# Autodesk Inventor assembly: carriage_assembly
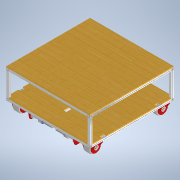
[picture p0: Inventor's stored thumbnail of the model, 180x180]
Saved by Autodesk Inventor 2021.3 (Build 253353000, 353)
## iProperties
Created: 2023-04-09
Part Number: carriage_assembly
Document SubType Name: Assembly
Designer: nxf77172
_SolveAssemblyDoc: Frame Generator Solve Assembly
_Version: 15.0.0
Author: nxf77172
## Documents named in this file (7)
- C:\Users\nxf77172\Desktop\mechanical_cleaned\custom_parts\carriage_assembly.iam
- C:\Users\nxf77172\Desktop\mechanical_cleaned\custom_parts\frame\frame_bottom.iam
- C:\Users\nxf77172\Desktop\mechanical_cleaned\custom_parts\drivetrain\drivetrain_assembly.iam
- C:\Users\nxf77172\Desktop\mechanical_cleaned\custom_parts\Bottom_Plate.ipt
- C:\Users\nxf77172\Desktop\mechanical_cleaned\custom_parts\frame\vertical_struts_frame.ipt
- C:\Users\nxf77172\Desktop\mechanical_cleaned\custom_parts\carriage_assembly\Frame\vertical_frame.iam
- C:\Users\nxf77172\Desktop\mechanical_cleaned\custom_parts\frame\frame_top.iam
## Components (9 placed, 6 different names)
1. frame_bottom:1 [sub-assembly] — Mate:1, Angle:1, Flush:1, Mate:2, Mate:3, Mate:4, Mate:5, Angle:2, Mate:7, Mate:8, Mate:10, Mate:11, Angle:3, Mate:12, Mate:13, Mate:15, Mate:16, Mate:20, Flush:2
2. drivetrain_assembly:1 [sub-assembly] — Mate:2, Mate:3, Mate:6
3. drivetrain_assembly:2 [sub-assembly] — Mate:7, Mate:8, Mate:9
4. drivetrain_assembly:3 [sub-assembly] — Mate:12, Mate:13, Mate:14
5. drivetrain_assembly:4 [sub-assembly] — Mate:15, Mate:16, Mate:17
6. Bottom_Plate:1 — Mate:18, Mate:19, Mate:20
7. vertical_struts_frame:1 — Flush:2
8. vertical_frame:1 [sub-assembly] — Mate:21, Angle:4, Flush:3, Flush:4
9. frame_top:1 [sub-assembly] — Mate:22, Flush:3, Flush:4
## Relationships (30: Mate 22, Angle 4, Flush 4)
- Mate:1: frame_bottom:1
- Angle:1 (0 deg): frame_bottom:1
- Flush:1: frame_bottom:1
- Mate:2: frame_bottom:1 ↔ drivetrain_assembly:1
- Mate:3: frame_bottom:1 ↔ drivetrain_assembly:1
- Mate:4: frame_bottom:1
- Mate:5: frame_bottom:1
- Angle:2 (0 deg): frame_bottom:1
- Mate:6: drivetrain_assembly:1
- Mate:7: frame_bottom:1 ↔ drivetrain_assembly:2
- Mate:8: frame_bottom:1 ↔ drivetrain_assembly:2
- Mate:9: drivetrain_assembly:2
- Mate:10: frame_bottom:1
- Mate:11: frame_bottom:1
- Angle:3 (0 deg): frame_bottom:1
- Mate:12: frame_bottom:1 ↔ drivetrain_assembly:3
- Mate:13: frame_bottom:1 ↔ drivetrain_assembly:3
- Mate:14: drivetrain_assembly:3
- Mate:15: frame_bottom:1 ↔ drivetrain_assembly:4
- Mate:16: frame_bottom:1 ↔ drivetrain_assembly:4
- Mate:17: drivetrain_assembly:4
- Mate:18: Bottom_Plate:1
- Mate:19: Bottom_Plate:1
- Mate:20: frame_bottom:1 ↔ Bottom_Plate:1
- Flush:2: frame_bottom:1 ↔ vertical_struts_frame:1
- Mate:21: vertical_frame:1
- Angle:4 (0 deg): vertical_frame:1
- Mate:22: frame_top:1
- Flush:3: vertical_frame:1 ↔ frame_top:1
- Flush:4: vertical_frame:1 ↔ frame_top:1
